# Autodesk Inventor assembly: motor mount plate
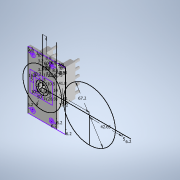
[picture p0: Inventor's stored thumbnail of the model, 180x180]
Saved by Autodesk Inventor 2022 (Build 260153000, 153)
## iProperties
Created: 2021-11-30
Part Number: motor mount plate
Document SubType Name: Assembly
Designer: a-dubs
Author: a-dubs
## Documents named in this file (3)
- S:\aw_gd\Coding and Projects\smart home\3d modelling\deadbolt controller\v3\motor mount plate.iam
- S:\aw_gd\Coding and Projects\smart home\3d modelling\deadbolt controller\v3\motor mount layer.ipt
- S:\aw_gd\Coding and Projects\smart home\3d modelling\deadbolt controller\v3\motor holder under.ipt
## Components (2 placed, 2 different names)
1. motor mount layer:1 — Mate:1, Flush:1, Flush:2
2. motor holder under:1 — Mate:1, Flush:1, Flush:2
## Relationships (3: Flush 2, Mate 1)
- Mate:1: motor mount layer:1 ↔ motor holder under:1
- Flush:1 (0.7 mm): motor mount layer:1 ↔ motor holder under:1
- Flush:2 (21 mm): motor mount layer:1 ↔ motor holder under:1
